# Autodesk Inventor assembly: Chappy
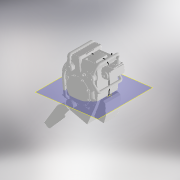
[picture p0: Inventor's stored thumbnail of the model, 180x180]
Saved by Autodesk Inventor 2022 (Build 260153000, 153)
## iProperties
Created: 2022-02-25
Part Number: Chappy
Document SubType Name: Assembly
Designer: joshw
Author: joshw
## Documents named in this file (4)
- C:\Users\joshw\Desktop\fun\Chappy.iam
- C:\Users\joshw\Desktop\man.ipt
- C:\Users\joshw\Desktop\NEW.ipt
- C:\Users\joshw\Desktop\fun\Head.ipt
## Components (3 placed, 3 different names)
1. man:1 — Mate:1, Mate:2
2. NEW:1 — Mate:1, Mate:2, Mate:3, Mate:4
3. Head:1 — Mate:3, Mate:4, Flush:1
## Relationships (5: Mate 4, Flush 1)
- Mate:1: man:1 ↔ NEW:1
- Mate:2: man:1 ↔ NEW:1
- Mate:3: NEW:1 ↔ Head:1
- Mate:4: NEW:1 ↔ Head:1
- Flush:1: Head:1
